# Autodesk Inventor assembly: сервы
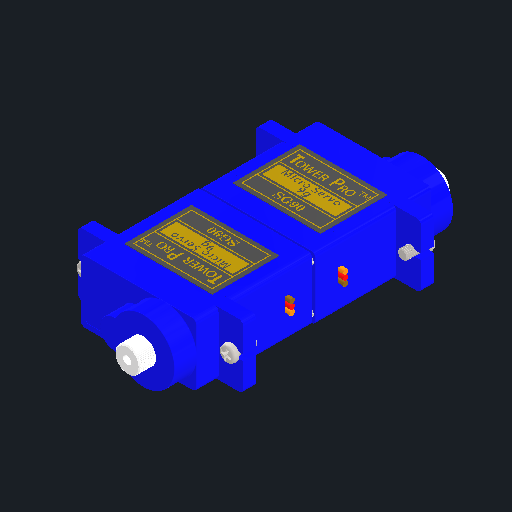
[picture p0: Inventor's stored thumbnail of the model, 512x512]
Saved by Autodesk Inventor 2022 (Build 260153000, 153)
## iProperties
Created: 2025-02-01
Part Number: сервы
Document SubType Name: Assembly
Designer: it
Author: it
## Documents named in this file (3)
- E:\машина\сервы.iam
- E:\abuyz lkz vfibyrb\SG90 - Micro Servo 9g - Tower Pro.1_Pea.ipt
- E:\abuyz lkz vfibyrb\SG90 - Micro Servo 9g - Tower Pro.6_BS EN ISO 7045 - M2 x 4 - Z - 4S.ipt
## Components (6 placed, 2 different names)
1. SG90 - Micro Servo 9g - Tower Pro.1_Pea:1
2. SG90 - Micro Servo 9g - Tower Pro.1_Pea:2
3. SG90 - Micro Servo 9g - Tower Pro.6_BS EN ISO 7045 - M2 x 4 - Z - 4S:1
4. SG90 - Micro Servo 9g - Tower Pro.6_BS EN ISO 7045 - M2 x 4 - Z - 4S:2
5. SG90 - Micro Servo 9g - Tower Pro.6_BS EN ISO 7045 - M2 x 4 - Z - 4S:3
6. SG90 - Micro Servo 9g - Tower Pro.6_BS EN ISO 7045 - M2 x 4 - Z - 4S:4
## Relationships (8: Mate 8)
- [Mate]: SG90 - Micro Servo 9g - Tower Pro.1_Pea:2 ↔ SG90 - Micro Servo 9g - Tower Pro.6_BS EN ISO 7045 - M2 x 4 - Z - 4S:2
- [Mate]: SG90 - Micro Servo 9g - Tower Pro.1_Pea:2 ↔ SG90 - Micro Servo 9g - Tower Pro.6_BS EN ISO 7045 - M2 x 4 - Z - 4S:2
- [Mate]: SG90 - Micro Servo 9g - Tower Pro.1_Pea:2 ↔ SG90 - Micro Servo 9g - Tower Pro.6_BS EN ISO 7045 - M2 x 4 - Z - 4S:1
- [Mate]: SG90 - Micro Servo 9g - Tower Pro.1_Pea:2 ↔ SG90 - Micro Servo 9g - Tower Pro.6_BS EN ISO 7045 - M2 x 4 - Z - 4S:1
- [Mate]: SG90 - Micro Servo 9g - Tower Pro.1_Pea:1 ↔ SG90 - Micro Servo 9g - Tower Pro.6_BS EN ISO 7045 - M2 x 4 - Z - 4S:4
- [Mate]: SG90 - Micro Servo 9g - Tower Pro.1_Pea:1 ↔ SG90 - Micro Servo 9g - Tower Pro.6_BS EN ISO 7045 - M2 x 4 - Z - 4S:3
- [Mate]: SG90 - Micro Servo 9g - Tower Pro.1_Pea:1 ↔ SG90 - Micro Servo 9g - Tower Pro.6_BS EN ISO 7045 - M2 x 4 - Z - 4S:3
- [Mate]: SG90 - Micro Servo 9g - Tower Pro.1_Pea:1 ↔ SG90 - Micro Servo 9g - Tower Pro.6_BS EN ISO 7045 - M2 x 4 - Z - 4S:4
